# Autodesk Inventor assembly: 51110 Groefkogellager - 70 mm
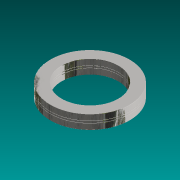
[picture p0: Inventor's stored thumbnail of the model, 180x180]
Saved by Autodesk Inventor 2020.2 (Build 242310000, 310)
## iProperties
Created: 2020-05-15
Part Number: 51110 Groefkogellager - 70 mm
Document SubType Name: Assembly
Designer: Svend
Author: Svend
## Documents named in this file (4)
- C:\Users\Svend\OneDrive\Documents\GitHub\BeerMinder\3D-model\bearings\51110 Groefkogellager - 70 mm.iam
- C:\Users\Svend\OneDrive\Documents\GitHub\BeerMinder\3D-model\bearings\ball.ipt
- C:\Users\Svend\OneDrive\Documents\GitHub\BeerMinder\3D-model\bearings\ballRing.ipt
- C:\Users\Svend\OneDrive\Documents\GitHub\BeerMinder\3D-model\bearings\UBC Bearing 51110 - buitenkant.ipt
## Components (22 placed, 3 different names)
1. ballRing:1 — Mate:1, Mate:2, Mate:3, Mate:4, Mate:5, Mate:6
2. UBC Bearing 51110 - buitenkant:1 — Mate:4, Mate:6
3. UBC Bearing 51110 - buitenkant:2 — Mate:3, Mate:5
4. ball:1 — Mate:1, Mate:2
5. ball:2
6. ball:3
7. ball:4
8. ball:5
9. ball:6
10. ball:7
11. ball:8
12. ball:9
13. ball:10
14. ball:11
15. ball:12
16. ball:13
17. ball:14
18. ball:15
19. ball:16
20. ball:17
21. ball:18
22. ball:19
## Component patterns: (19 elements, first: ball:1)
## Relationships (6: Mate 6)
- Mate:1: ballRing:1 ↔ ball:1
- Mate:2: ballRing:1 ↔ ball:1
- Mate:3: ballRing:1 ↔ UBC Bearing 51110 - buitenkant:2
- Mate:4: ballRing:1 ↔ UBC Bearing 51110 - buitenkant:1
- Mate:5 (0.2 mm): ballRing:1 ↔ UBC Bearing 51110 - buitenkant:2
- Mate:6 (0.2 mm): ballRing:1 ↔ UBC Bearing 51110 - buitenkant:1
